# Autodesk Inventor assembly: axishelix
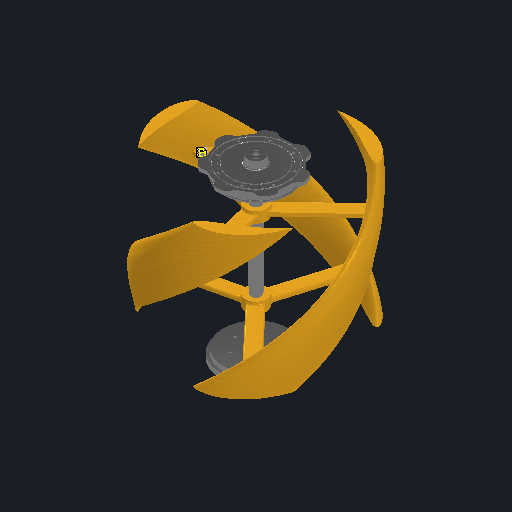
[picture p0: Inventor's stored thumbnail of the model, 512x512]
Saved by Autodesk Inventor 2025.4 (Build 294407000, 407)
## iProperties
Created: 2026-03-08
Part Number: axishelix
Document SubType Name: Assembly
Designer: danie
Author: danie
## Documents named in this file (5)
- C:\Users\danie\OneDrive\Documentos\Inventor\Arbol\V4\V4\axishelix.iam
- C:\Users\danie\OneDrive\Documentos\Inventor\Arbol\V4\V4\Vertical\Axis.ipt
- C:\Users\danie\OneDrive\Documentos\Inventor\Arbol\V4\V4\Vertical\FanWind.ipt
- C:\Users\danie\OneDrive\Documentos\Inventor\Arbol\V4\V4\Vertical\Soporte22.ipt
- C:\Users\danie\OneDrive\Documentos\Inventor\Arbol\V4\V4\Vertical\Tapa_Superior2.ipt
## Components (4 placed, 4 different names)
1. Axis:1 — Mate:1, Mate:2, Flush:1, Mate:3, Flush:2, Mate:6, Flush:3
2. FanWind:1 — Mate:3, Mate:5
3. Soporte22:1 — Mate:4, Flush:2, Mate:5
4. Tapa_Superior2:1 — Mate:6, Flush:3
## Relationships (9: Mate 6, Flush 3)
- Mate:1: Axis:1
- Mate:2: Axis:1
- Flush:1: Axis:1
- Mate:3: Axis:1 ↔ FanWind:1
- Mate:4: Soporte22:1
- Flush:2: Axis:1 ↔ Soporte22:1
- Mate:5: FanWind:1 ↔ Soporte22:1
- Mate:6: Axis:1 ↔ Tapa_Superior2:1
- Flush:3: Axis:1 ↔ Tapa_Superior2:1
